# Autodesk Inventor assembly: ShoulderJoint_Concept1_LightWeight_Assembly
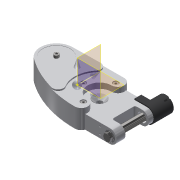
[picture p0: Inventor's stored thumbnail of the model, 180x180]
Saved by Autodesk Inventor 2021.4 (Build 254397000, 397)
## iProperties
Created: 2022-07-05
Part Number: ShoulderJoint_Concept1_LightWeight_Assembly
Material: Generisch
Document SubType Name: Assembly
Designer: alexw
Mass: 482.034 g
Surface Area: 624.028 cm^2
Volume: 214.647 cm^3
Density: 2.2457 g/cm^3
Author: alexw
## Documents named in this file (14)
- C:\Users\alexw\Documents\Inventor\Projects\03_CurrentProjects\MasterThesis\TrainingConsol_220422\Workgroups\Workgroup\ShoulderJoint_Concept1_LightWeight_Assembly.iam
- C:\Users\alexw\Documents\Inventor\Projects\03_CurrentProjects\MasterThesis\TrainingConsol_220422\Workgroups\Workgroup\Shoulder_Joint_v2.ipt
- C:\Users\alexw\Documents\Inventor\Projects\03_CurrentProjects\MasterThesis\TrainingConsol_220422\Workgroups\Workgroup\Shoulder_Joint_Yawn_Shaft.ipt
- C:\Users\alexw\Documents\Inventor\Projects\03_CurrentProjects\MasterThesis\TrainingConsol_220422\Workgroups\Workgroup\DIN EN ISO 4017 - M6 x 12.ipt
- C:\Users\alexw\Documents\Inventor\Projects\03_CurrentProjects\MasterThesis\TrainingConsol_220422\Workgroups\Workgroup\W 61700 X-2RS1.iam
- C:\Users\alexw\Documents\Inventor\Projects\03_CurrentProjects\MasterThesis\TrainingConsol_220422\Workgroups\Workgroup\DIN 988 - 6 x 12 x 0,5.ipt
- C:\Users\alexw\Documents\Inventor\Projects\03_CurrentProjects\MasterThesis\TrainingConsol_220422\Workgroups\Workgroup\Shoulder_Yawn_Sensor_Connector.ipt
- C:\Users\alexw\Documents\Inventor\Projects\03_CurrentProjects\MasterThesis\TrainingConsol_220422\Workgroups\Workgroup\Magnetic Encoder.ipt
- C:\Users\alexw\Documents\Inventor\Projects\03_CurrentProjects\MasterThesis\TrainingConsol_220422\Workgroups\Workgroup\DIN EN ISO 4762 - M2 x 6.ipt
- C:\Users\alexw\Documents\Inventor\Projects\03_CurrentProjects\MasterThesis\TrainingConsol_220422\Workgroups\Workgroup\DIN EN ISO 4762 - M2 x 12.ipt
- C:\Users\alexw\Documents\Inventor\Projects\03_CurrentProjects\MasterThesis\TrainingConsol_220422\Workgroups\Workgroup\ContentCenter\en-US\ISO 4762(2)\ISO 4762 - M4 x 6ISO.ipt
- C:\Users\alexw\Documents\Inventor\Projects\03_CurrentProjects\MasterThesis\TrainingConsol_220422\Workgroups\Workgroup\CounterWeightFixation_oldVersion.ipt
- C:\Users\alexw\Documents\Inventor\Projects\03_CurrentProjects\MasterThesis\TrainingConsol_220422\Workgroups\Workgroup\CounterWeights_Brass.ipt
- C:\Users\alexw\Documents\Inventor\Projects\03_CurrentProjects\MasterThesis\TrainingConsol_220422\Workgroups\Workgroup\ContentCenter\en-US\ISO 4762(2)\ISO 4762 - M4 x 10ISO.ipt
## Components (20 placed, 13 different names)
1. Shoulder_Joint_v2:1 — Mate:27, Mate:28, Mate:29, Mate:30, Flush:3, Flush:4, Mate:37, Mate:39, Mate:41
2. Shoulder_Joint_Yawn_Shaft:1
3. DIN EN ISO 4017 M6 x 12:1
4. W 61700 X-2RS1:1 [sub-assembly]
5. W 61700 X-2RS1:2 [sub-assembly]
6. W 61700 X-2RS1:3 [sub-assembly] — Mate:27
7. W 61700 X-2RS1:4 [sub-assembly]
8. DIN 988 6 x 12 x 0,5:1
9. Shoulder_Yawn_Sensor_Connector:1
10. Magnetic Encoder:1
11. DIN EN ISO 4762 M2 x 6:1
12. DIN EN ISO 4762 M2 x 6:2
13. DIN EN ISO 4762 M2 x 12:1
14. DIN EN ISO 4762 M2 x 12:2
15. CounterWeightFixation_oldVersion:1 — Mate:28, Mate:29, Mate:38, Mate:40, Mate:42, Mate:44, Mate:45, Mate:46, Mate:48
16. ISO 4762 M4 x 6:1 — Mate:37, Mate:38
17. ISO 4762 M4 x 6:2 — Mate:39, Mate:40
18. ISO 4762 M4 x 6:3 — Mate:41, Mate:42, Mate:44
19. CounterWeights_Brass:1 — Mate:45, Mate:46, Mate:47
20. ISO 4762 M4 x 10:1 — Mate:47, Mate:48
## Relationships (44: Mate 40, Flush 4)
- [Mate]: Shoulder_Joint_Yawn_Shaft:1 ↔ DIN EN ISO 4017 M6 x 12:1
- [Mate]: W 61700 X-2RS1:1 ↔ W 61700 X-2RS1:2
- [Mate]: W 61700 X-2RS1:1 ↔ W 61700 X-2RS1:2
- [Mate]: W 61700 X-2RS1:3 ↔ W 61700 X-2RS1:4
- [Mate]: W 61700 X-2RS1:3 ↔ W 61700 X-2RS1:4
- [Mate]: Shoulder_Joint_Yawn_Shaft:1 ↔ W 61700 X-2RS1:2
- [Mate]: DIN EN ISO 4017 M6 x 12:1 ↔ DIN 988 6 x 12 x 0,5:1
- [Mate]: W 61700 X-2RS1:3 ↔ DIN 988 6 x 12 x 0,5:1
- [Mate]: DIN EN ISO 4017 M6 x 12:1 ↔ DIN 988 6 x 12 x 0,5:1
- [Mate]: Shoulder_Joint_Yawn_Shaft:1 ↔ Shoulder_Yawn_Sensor_Connector:1
- [Mate]: Shoulder_Yawn_Sensor_Connector:1 ↔ Magnetic Encoder:1
- [Mate]: Shoulder_Yawn_Sensor_Connector:1 ↔ Magnetic Encoder:1
- [Mate]: Shoulder_Yawn_Sensor_Connector:1 ↔ Magnetic Encoder:1
- [Mate]: Shoulder_Yawn_Sensor_Connector:1 ↔ DIN EN ISO 4762 M2 x 6:1
- [Mate]: Magnetic Encoder:1 ↔ DIN EN ISO 4762 M2 x 6:1
- [Mate]: Shoulder_Yawn_Sensor_Connector:1 ↔ DIN EN ISO 4762 M2 x 6:2
- [Mate]: Magnetic Encoder:1 ↔ DIN EN ISO 4762 M2 x 6:2
- [Mate]: Shoulder_Yawn_Sensor_Connector:1 ↔ DIN EN ISO 4762 M2 x 12:1
- [Mate]: Shoulder_Yawn_Sensor_Connector:1 ↔ DIN EN ISO 4762 M2 x 12:2
- [Mate]: Shoulder_Joint_Yawn_Shaft:1 ↔ W 61700 X-2RS1:4
- [Mate]: Shoulder_Joint_v2:1 ↔ Shoulder_Yawn_Sensor_Connector:1
- [Flush]: Shoulder_Joint_v2:1 ↔ W 61700 X-2RS1:3
- [Mate]: Shoulder_Joint_v2:1 ↔ Shoulder_Yawn_Sensor_Connector:1
- [Flush]: Shoulder_Joint_v2:1 ↔ W 61700 X-2RS1:2
- [Mate]: Shoulder_Joint_Yawn_Shaft:1 ↔ W 61700 X-2RS1:2
- [Mate]: Shoulder_Joint_v2:1 ↔ DIN EN ISO 4762 M2 x 12:2
- [Mate]: Shoulder_Joint_v2:1 ↔ DIN EN ISO 4762 M2 x 12:1
- Mate:27: Shoulder_Joint_v2:1 ↔ W 61700 X-2RS1:3
- Mate:28: Shoulder_Joint_v2:1 ↔ CounterWeightFixation_oldVersion:1
- Mate:29: Shoulder_Joint_v2:1 ↔ CounterWeightFixation_oldVersion:1
- Mate:30: Shoulder_Joint_v2:1
- Flush:3: Shoulder_Joint_v2:1
- Flush:4: Shoulder_Joint_v2:1
- Mate:37: Shoulder_Joint_v2:1 ↔ ISO 4762 M4 x 6:1
- Mate:38: CounterWeightFixation_oldVersion:1 ↔ ISO 4762 M4 x 6:1
- Mate:39: Shoulder_Joint_v2:1 ↔ ISO 4762 M4 x 6:2
- Mate:40: CounterWeightFixation_oldVersion:1 ↔ ISO 4762 M4 x 6:2
- Mate:41: Shoulder_Joint_v2:1 ↔ ISO 4762 M4 x 6:3
- Mate:42: CounterWeightFixation_oldVersion:1 ↔ ISO 4762 M4 x 6:3
- Mate:44: CounterWeightFixation_oldVersion:1 ↔ ISO 4762 M4 x 6:3
- Mate:45: CounterWeightFixation_oldVersion:1 ↔ CounterWeights_Brass:1
- Mate:46: CounterWeightFixation_oldVersion:1 ↔ CounterWeights_Brass:1
- Mate:47: CounterWeights_Brass:1 ↔ ISO 4762 M4 x 10:1
- Mate:48: CounterWeightFixation_oldVersion:1 ↔ ISO 4762 M4 x 10:1
